# Autodesk Inventor assembly: Beta Motor Assembly
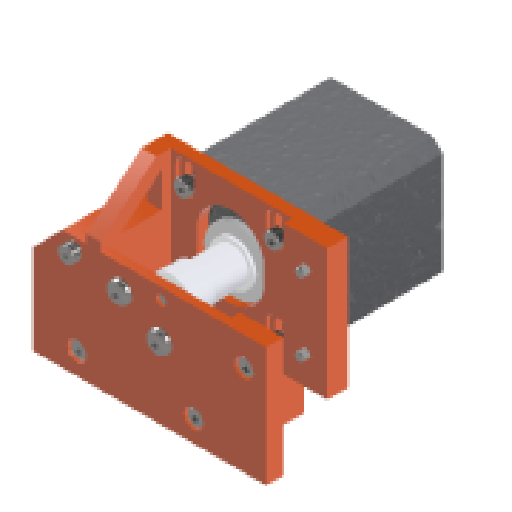
[picture p0: Inventor's stored thumbnail of the model, 512x512]
Saved by Autodesk Inventor 2023.2 (Build 272271000, 271)
## iProperties
Created: 2023-02-03
Part Number: Beta Motor Assembly
Document SubType Name: Assembly
Designer: remop
Author: remop
## Documents named in this file (8)
- C:\Users\remop\OneDrive\Documents\Inventor\3D Printers\LuEVO\Mk5_FullKinematic\Beta Motor Assembly.iam
- C:\Users\remop\OneDrive\Documents\Inventor\3D Printers\LuEVO\Mk5_FullKinematic\Beta Motor Mount.ipt
- C:\Users\remop\OneDrive\Documents\Inventor\3D Printers\LuEVO\Mk5_FullKinematic\XY Axis Motor (Stepper).ipt
- C:\Users\remop\OneDrive\Documents\Inventor\3D Printers\LuEVO\Mk5_FullKinematic\Belt Pulley.ipt
- C:\Users\remop\OneDrive\Documents\Inventor\3D Printers\LuEVO\Mk5_FullKinematic\Alpha Idler Top.ipt
- C:\Users\remop\OneDrive\Documents\Inventor\Content Center Files\R2023\en-US\AS 1420\AS 1420 - 1973 - M3 x 6.ipt
- C:\Users\remop\OneDrive\Documents\Inventor\Content Center Files\R2023\en-US\AS 1420\AS 1420 - 1973 - M3 x 12.ipt
- C:\Users\remop\OneDrive\Documents\Inventor\Content Center Files\R2023\en-US\BS 4168(6)\BS 4168 - M4 x 8(6).ipt
## Components (18 placed, 7 different names)
1. Beta Motor Mount:1 — Rigid:3, Flush:1, Flush:2, Mate:1, Insert:4, Insert:5, Insert:6, Insert:7, Insert:8, Insert:11, Insert:13, Insert:15
2. XY Axis Motor (Stepper):1 — Rigid:2, Rigid:3
3. Belt Pulley:1 — Rigid:2
4. Alpha Idler Top:1 — Flush:1, Flush:2, Mate:1, Insert:1, Insert:2, Insert:3, Mate:2, Mate:3, Insert:16, Insert:17
5. AS 1420 - Metric M3 x 6:1 — Insert:1
6. AS 1420 - Metric M3 x 6:2 — Insert:2
7. AS 1420 - Metric M3 x 6:3 — Insert:3
8. AS 1420 - Metric M3 x 6:4 — Insert:4
9. AS 1420 - Metric M3 x 6:5 — Insert:5
10. AS 1420 - Metric M3 x 6:6 — Insert:6
11. AS 1420 - Metric M3 x 6:7 — Insert:7
12. AS 1420 - Metric M3 x 6:8 — Insert:8
13. AS 1420 - Metric M3 x 6:11 — Insert:11
14. AS 1420 - Metric M3 x 6:13 — Insert:13
15. AS 1420 - Metric M3 x 6:15 — Insert:15
16. AS 1420 - Metric M3 x 12:1 — Mate:2, Mate:3
17. BS 4168 : Part 6 Hexagon socket countersunk and button head screws - Metric series - Metric M4 x 8:1 — Insert:16
18. BS 4168 : Part 6 Hexagon socket countersunk and button head screws - Metric series - Metric M4 x 8:2 — Insert:17
## Relationships (20: Insert 13, Mate 3, WeldJoint 2, Flush 2)
- Rigid:2 [WeldJoint] (-0.5 mm): XY Axis Motor (Stepper):1 ↔ Belt Pulley:1
- Rigid:3 [WeldJoint]: Beta Motor Mount:1 ↔ XY Axis Motor (Stepper):1
- Flush:1: Beta Motor Mount:1 ↔ Alpha Idler Top:1
- Flush:2: Beta Motor Mount:1 ↔ Alpha Idler Top:1
- Mate:1 (15 mm): Beta Motor Mount:1 ↔ Alpha Idler Top:1
- Insert:1: Alpha Idler Top:1 ↔ AS 1420 - Metric M3 x 6:1
- Insert:2: Alpha Idler Top:1 ↔ AS 1420 - Metric M3 x 6:2
- Insert:3: Alpha Idler Top:1 ↔ AS 1420 - Metric M3 x 6:3
- Insert:4: Beta Motor Mount:1 ↔ AS 1420 - Metric M3 x 6:4
- Insert:5: Beta Motor Mount:1 ↔ AS 1420 - Metric M3 x 6:5
- Insert:6: Beta Motor Mount:1 ↔ AS 1420 - Metric M3 x 6:6
- Insert:7: Beta Motor Mount:1 ↔ AS 1420 - Metric M3 x 6:7
- Insert:8: Beta Motor Mount:1 ↔ AS 1420 - Metric M3 x 6:8
- Insert:11: Beta Motor Mount:1 ↔ AS 1420 - Metric M3 x 6:11
- Insert:13: Beta Motor Mount:1 ↔ AS 1420 - Metric M3 x 6:13
- Insert:15: Beta Motor Mount:1 ↔ AS 1420 - Metric M3 x 6:15
- Mate:2: Alpha Idler Top:1 ↔ AS 1420 - Metric M3 x 12:1
- Mate:3: Alpha Idler Top:1 ↔ AS 1420 - Metric M3 x 12:1
- Insert:16: Alpha Idler Top:1 ↔ BS 4168 : Part 6 Hexagon socket countersunk and button head screws - Metric series - Metric M4 x 8:1
- Insert:17: Alpha Idler Top:1 ↔ BS 4168 : Part 6 Hexagon socket countersunk and button head screws - Metric series - Metric M4 x 8:2
